# Autodesk Inventor assembly: enc-FrontPanel Unten - Assembly no Absorber
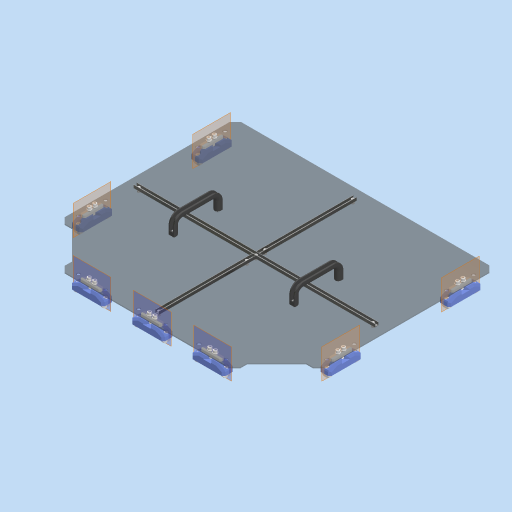
[picture p0: Inventor's stored thumbnail of the model, 512x512]
Saved by Autodesk Inventor 2023.2 (Build 272271000, 271)
## iProperties
Created: 2023-11-30
Part Number: enc-FrontPanel Unten - Assembly no Absorber
Document SubType Name: Assembly
Designer: Nils Bade
Author: Nils Bade
## Documents named in this file (8)
- C:\Users\nilsb\Documents\Inventor\Projektarbeit-Bade\Enclosure\enc-FrontPanel Unten - Assembly no Absorber.iam
- C:\Users\nilsb\Documents\Inventor\Projektarbeit-Bade\Enclosure\Magnet PanelFrame Straight connected.iam
- C:\Users\nilsb\Documents\Inventor\Projektarbeit-Bade\Enclosure\U-Profil PanelSupport 10x8x660mm.ipt
- C:\Users\nilsb\Documents\Inventor\Projektarbeit-Bade\Enclosure\U-Profil PanelSupport 10x8x265mm.ipt
- C:\Users\nilsb\Documents\Inventor\Projektarbeit-Bade\Schrauben\Cap Head Screw M4x8 - DIN912.ipt
- C:\Users\nilsb\Documents\Inventor\Projektarbeit-Bade\RatRig_Standards\Hex Nut - M4 DIN934.ipt
- C:\Users\nilsb\Documents\Inventor\Projektarbeit-Bade\Enclosure\enc-FrontPanel Unten.ipt
- C:\Users\nilsb\Documents\Inventor\Projektarbeit-Bade\Enclosure\item_Handgriff_PA120_Assembly.iam
## Components (27 placed, 6 different names)
1. enc-FrontPanel Unten 597x710:1 — Passend:81, Passend:82, Passend:83, Passend:84, Passend:85, Passend:86
2. Magnet PanelFrame Straight connected:1 [sub-assembly]
3. Magnet PanelFrame Straight connected:2 [sub-assembly]
4. Magnet PanelFrame Straight connected:3 [sub-assembly]
5. Magnet PanelFrame Straight connected:4 [sub-assembly]
6. Magnet PanelFrame Straight connected:5 [sub-assembly]
7. Magnet PanelFrame Straight connected:6 [sub-assembly]
8. Magnet PanelFrame Straight connected:7 [sub-assembly]
9. U-Profil PanelSupport 10x8x265mm:1 — Passend:54, Passend:62, Passend:65
10. U-Profil PanelSupport 10x8x265mm:2 — Passend:61, Passend:66
11. U-Profil PanelSupport 10x8x265mm:3 — Passend:63, Passend:64
12. Cap Head Screw M4x8 - DIN912:1 — Passend:54, Passend:73
13. Cap Head Screw M4x8 - DIN912:2 — Passend:63, Passend:71
14. Cap Head Screw M4x8 - DIN912:3 — Passend:65, Passend:72
15. Cap Head Screw M4x8 - DIN912:4 — Passend:61, Passend:69
16. Cap Head Screw M4x8 - DIN912:5 — Passend:66, Passend:67
17. Cap Head Screw M4x8 - DIN912:6 — Passend:62, Passend:70
18. Cap Head Screw M4x8 - DIN912:7 — Passend:64, Passend:75
19. Hex Nut - M4 DIN934:1 — Passend:67
20. Hex Nut - M4 DIN934:2 — Passend:69
21. Hex Nut - M4 DIN934:3 — Passend:70
22. Hex Nut - M4 DIN934:4 — Passend:71
23. Hex Nut - M4 DIN934:5 — Passend:75
24. Hex Nut - M4 DIN934:6 — Passend:72
25. Hex Nut - M4 DIN934:7 — Passend:73
26. item_Handgriff_120er:1 [sub-assembly] — Passend:81, Passend:83, Passend:86
27. item_Handgriff_120er:2 [sub-assembly] — Passend:82, Passend:84, Passend:85
## Relationships (64: Mate 64)
- [Mate]: enc-FrontPanel Unten 597x710:1 ↔ Magnet PanelFrame Straight connected:5
- [Mate]: enc-FrontPanel Unten 597x710:1 ↔ Magnet PanelFrame Straight connected:5
- [Mate]: enc-FrontPanel Unten 597x710:1 ↔ Magnet PanelFrame Straight connected:5
- [Mate]: enc-FrontPanel Unten 597x710:1 ↔ Magnet PanelFrame Straight connected:6
- [Mate]: enc-FrontPanel Unten 597x710:1 ↔ Magnet PanelFrame Straight connected:6
- [Mate]: enc-FrontPanel Unten 597x710:1 ↔ Magnet PanelFrame Straight connected:6
- [Mate]: enc-FrontPanel Unten 597x710:1 ↔ Magnet PanelFrame Straight connected:7
- [Mate]: enc-FrontPanel Unten 597x710:1 ↔ Magnet PanelFrame Straight connected:7
- [Mate]: enc-FrontPanel Unten 597x710:1 ↔ Magnet PanelFrame Straight connected:7
- [Mate]: enc-FrontPanel Unten 597x710:1 ↔ Magnet PanelFrame Straight connected:2
- [Mate]: enc-FrontPanel Unten 597x710:1 ↔ Magnet PanelFrame Straight connected:2
- [Mate]: enc-FrontPanel Unten 597x710:1 ↔ Magnet PanelFrame Straight connected:2
- [Mate]: enc-FrontPanel Unten 597x710:1 ↔ Magnet PanelFrame Straight connected:1
- [Mate]: enc-FrontPanel Unten 597x710:1 ↔ Magnet PanelFrame Straight connected:1
- [Mate]: enc-FrontPanel Unten 597x710:1 ↔ Magnet PanelFrame Straight connected:1
- [Mate]: enc-FrontPanel Unten 597x710:1 ↔ Magnet PanelFrame Straight connected:3
- [Mate]: enc-FrontPanel Unten 597x710:1 ↔ Magnet PanelFrame Straight connected:3
- [Mate]: enc-FrontPanel Unten 597x710:1 ↔ Magnet PanelFrame Straight connected:4
- [Mate]: enc-FrontPanel Unten 597x710:1 ↔ Magnet PanelFrame Straight connected:4
- [Mate]: enc-FrontPanel Unten 597x710:1 ↔ Magnet PanelFrame Straight connected:4
- [Mate]: enc-FrontPanel Unten 597x710:1 ↔ Magnet PanelFrame Straight connected:3
- [Mate]: enc-FrontPanel Unten 597x710:1 ↔ U-Profil PanelSupport 10x8x265mm:1
- [Mate]: enc-FrontPanel Unten 597x710:1 ↔ U-Profil PanelSupport 10x8x265mm:1
- [Mate]: enc-FrontPanel Unten 597x710:1 ↔ U-Profil PanelSupport 10x8x265mm:1
- [Mate]: enc-FrontPanel Unten 597x710:1 ↔ U-Profil PanelSupport 10x8x265mm:3
- [Mate]: enc-FrontPanel Unten 597x710:1 ↔ U-Profil PanelSupport 10x8x265mm:3
- [Mate]: enc-FrontPanel Unten 597x710:1 ↔ U-Profil PanelSupport 10x8x265mm:3
- [Mate]: enc-FrontPanel Unten 597x710:1 ↔ U-Profil PanelSupport 10x8x265mm:2
- [Mate]: enc-FrontPanel Unten 597x710:1 ↔ U-Profil PanelSupport 10x8x265mm:2
- [Mate]: enc-FrontPanel Unten 597x710:1 ↔ U-Profil PanelSupport 10x8x265mm:2
- [Mate]: enc-FrontPanel Unten 597x710:1 ↔ Cap Head Screw M4x8 - DIN912:1
- Passend:54 [Mate]: U-Profil PanelSupport 10x8x265mm:1 ↔ Cap Head Screw M4x8 - DIN912:1
- [Mate]: enc-FrontPanel Unten 597x710:1 ↔ Cap Head Screw M4x8 - DIN912:7
- [Mate]: enc-FrontPanel Unten 597x710:1 ↔ Cap Head Screw M4x8 - DIN912:2
- [Mate]: enc-FrontPanel Unten 597x710:1 ↔ Cap Head Screw M4x8 - DIN912:6
- [Mate]: enc-FrontPanel Unten 597x710:1 ↔ Cap Head Screw M4x8 - DIN912:4
- [Mate]: enc-FrontPanel Unten 597x710:1 ↔ Cap Head Screw M4x8 - DIN912:3
- [Mate]: enc-FrontPanel Unten 597x710:1 ↔ Cap Head Screw M4x8 - DIN912:5
- Passend:61 [Mate]: U-Profil PanelSupport 10x8x265mm:2 ↔ Cap Head Screw M4x8 - DIN912:4
- Passend:62 [Mate]: U-Profil PanelSupport 10x8x265mm:1 ↔ Cap Head Screw M4x8 - DIN912:6
- Passend:63 [Mate]: U-Profil PanelSupport 10x8x265mm:3 ↔ Cap Head Screw M4x8 - DIN912:2
- Passend:64 [Mate]: U-Profil PanelSupport 10x8x265mm:3 ↔ Cap Head Screw M4x8 - DIN912:7
- Passend:65 [Mate]: U-Profil PanelSupport 10x8x265mm:1 ↔ Cap Head Screw M4x8 - DIN912:3
- Passend:66 [Mate]: U-Profil PanelSupport 10x8x265mm:2 ↔ Cap Head Screw M4x8 - DIN912:5
- Passend:67 [Mate]: Cap Head Screw M4x8 - DIN912:5 ↔ Hex Nut - M4 DIN934:1
- [Mate]: enc-FrontPanel Unten 597x710:1 ↔ Hex Nut - M4 DIN934:1
- Passend:69 [Mate]: Cap Head Screw M4x8 - DIN912:4 ↔ Hex Nut - M4 DIN934:2
- Passend:70 [Mate]: Cap Head Screw M4x8 - DIN912:6 ↔ Hex Nut - M4 DIN934:3
- Passend:71 [Mate]: Cap Head Screw M4x8 - DIN912:2 ↔ Hex Nut - M4 DIN934:4
- Passend:72 [Mate]: Cap Head Screw M4x8 - DIN912:3 ↔ Hex Nut - M4 DIN934:6
- Passend:73 [Mate]: Cap Head Screw M4x8 - DIN912:1 ↔ Hex Nut - M4 DIN934:7
- [Mate]: enc-FrontPanel Unten 597x710:1 ↔ Hex Nut - M4 DIN934:5
- Passend:75 [Mate]: Cap Head Screw M4x8 - DIN912:7 ↔ Hex Nut - M4 DIN934:5
- [Mate]: enc-FrontPanel Unten 597x710:1 ↔ Hex Nut - M4 DIN934:4
- [Mate]: enc-FrontPanel Unten 597x710:1 ↔ Hex Nut - M4 DIN934:6
- [Mate]: enc-FrontPanel Unten 597x710:1 ↔ Hex Nut - M4 DIN934:2
- [Mate]: enc-FrontPanel Unten 597x710:1 ↔ Hex Nut - M4 DIN934:3
- [Mate]: enc-FrontPanel Unten 597x710:1 ↔ Hex Nut - M4 DIN934:7
- Passend:81 [Mate]: enc-FrontPanel Unten 597x710:1 ↔ item_Handgriff_120er:1
- Passend:82 [Mate]: enc-FrontPanel Unten 597x710:1 ↔ item_Handgriff_120er:2
- Passend:83 [Mate]: enc-FrontPanel Unten 597x710:1 ↔ item_Handgriff_120er:1
- Passend:84 [Mate]: enc-FrontPanel Unten 597x710:1 ↔ item_Handgriff_120er:2
- Passend:85 [Mate]: enc-FrontPanel Unten 597x710:1 ↔ item_Handgriff_120er:2
- Passend:86 [Mate]: enc-FrontPanel Unten 597x710:1 ↔ item_Handgriff_120er:1
